# Autodesk Inventor assembly: 206.001.01_Schieberbetaetigung
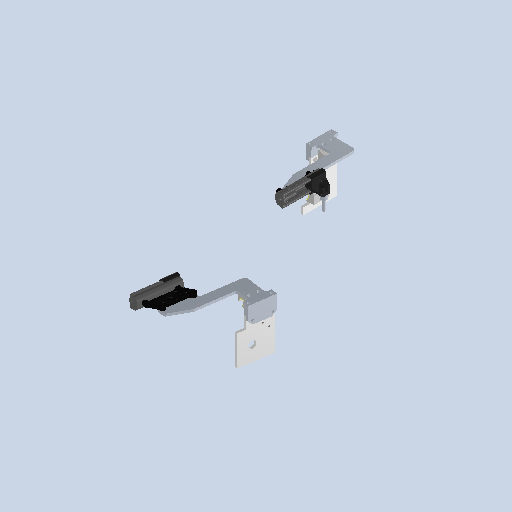
[picture p0: Inventor's stored thumbnail of the model, 512x512]
Saved by Autodesk Inventor 2022 (Build 260153000, 153)
## iProperties
Created: 2021-11-14
Part Number: 206.001.01_Schieberbetaetigung
Document SubType Name: Assembly
Designer: Oliver Ungerer
KODE_ZEICHNUNGSNUMMER: TFVEM_110M
BENENNUNG: Fuehrung Schieber
BEARBEITER_NAME: Ungerer O.
MASSE: 2.190774
PDMREV: 0.0+
PDMRL: Entwicklung
PROI_REVISION: 0
PROI_VERSION: 0+
PROI_RELEASE: Entwicklung
PTC_MODIFIED: True
PROI_CREATED_BY: Kantioler_adm
PROI_CREATED_ON: 07.03.2008 12:11:19
PROI_LOCATION: Root-Ordner/Pro_stds/Start_Files
MATERIALART: -
EINHEIT: ST
HERSTELLER_PREIS: 0.0
PRUEFER_NAME: Uo
PTC_ORGANIZATION_ID: Durst
PTC_WM_REVISION: 0
PTC_WM_ITERATION: 0
PTC_WM_VERSION: 0.0
PTC_WM_LIFECYCLE_STATE: Entwicklung
PTC_WM_LIFECYCLE: 02 Durst
PTC_WM_CREATED_BY: Oliver Ungerer (oungerer: Durst)
PTC_WM_CREATED_ON: 01.08.21
PTC_WM_MODIFIED_BY: Oliver Ungerer (oungerer: Durst)
PTC_WM_MODIFIED_ON: 01.08.21
AEND_INDEX: 0
VERSION: 0
STATUS: 0.0
Author: Oliver Ungerer
## Documents named in this file (11)
- C:\Users\kaebi\OneDrive - mci4me.at\03_MCI Master\4.Semester_SS2022\Masterarbeit\Software\CAD_TeachingFactory\206.002.01_Schieberbetaetigung.iam
- C:\Users\kaebi\OneDrive - mci4me.at\03_MCI Master\4.Semester_SS2022\Masterarbeit\Software\CAD_TeachingFactory\106.016.01_Schienenfuehrung.ipt
- C:\Users\kaebi\OneDrive - mci4me.at\03_MCI Master\4.Semester_SS2022\Masterarbeit\Software\CAD_TeachingFactory\106.019.01_Distanzplatte.ipt
- C:\Users\kaebi\OneDrive - mci4me.at\03_MCI Master\4.Semester_SS2022\Masterarbeit\Software\CAD_TeachingFactory\106.018.01_Schieberelement_oben.ipt
- C:\Users\kaebi\OneDrive - mci4me.at\03_MCI Master\4.Semester_SS2022\Masterarbeit\Software\CAD_TeachingFactory\106.020.01_Winkelaufnahme_Schwert_unten.ipt
- C:\Users\kaebi\OneDrive - mci4me.at\03_MCI Master\4.Semester_SS2022\Masterarbeit\Software\CAD_TeachingFactory\106.030.01_Schwert_oben.ipt
- C:\Users\kaebi\OneDrive - mci4me.at\03_MCI Master\4.Semester_SS2022\Masterarbeit\Software\CAD_TeachingFactory\106.033.01_Schwert_unten.ipt
- C:\Users\kaebi\OneDrive - mci4me.at\03_MCI Master\4.Semester_SS2022\Masterarbeit\Software\CAD_TeachingFactory\206.003.02_Kraftlimitierung.iam
- C:\Users\kaebi\OneDrive - mci4me.at\03_MCI Master\4.Semester_SS2022\Masterarbeit\Software\CAD_TeachingFactory\206.004.02_Kraftlimitierung.iam
- C:\Users\kaebi\OneDrive - mci4me.at\03_MCI Master\4.Semester_SS2022\Masterarbeit\Software\CAD_TeachingFactory\106.035.01_Distanzbolzen_gross.ipt
- C:\Users\kaebi\OneDrive - mci4me.at\03_MCI Master\4.Semester_SS2022\Masterarbeit\Software\CAD_TeachingFactory\106.034.01_Schieberelement_unten.ipt
## Components (15 placed, 10 different names)
1. 106.019.01_Distanzplatte — Passend:18, Passend:29, Passend:77, Passend:78, Passend:79
2. 106.019.01_Distanzplatte:1 — Passend:26, Passend:75, Passend:76, Passend:100, Passend:101
3. 106.035.01_Distanzbolzen_gross — Passend:59, Passend:60
4. 106.016.01_Schienenfuehrung:5 — Passend:97
5. 106.016.01_Schienenfuehrung:6 — Passend:98, Passend:99
6. 106.034.01_Schieberelement_unten:2 — Passend:97, Passend:98, Passend:99
7. 106.020.01_Winkelaufnahme_Schwert_unten:3
8. 106.033.01_Schwert_unten:2
9. 206.003.02_Kraftlimitierung:2 [sub-assembly]
10. 106.016.01_Schienenfuehrung — Passend:18, Passend:77, Passend:78
11. 106.016.01_Schienenfuehrung:1 — Passend:26, Passend:75, Passend:76, Passend:80
12. 106.018.01_Schieberelement_oben — Passend:29, Passend:36, Passend:37, Passend:38, Passend:50, Passend:79, Passend:80, Passend:83, Passend:84, Passend:100, Passend:101
13. 106.020.01_Winkelaufnahme_Schwert_unten — Passend:36, Passend:37, Passend:38, Passend:42, Passend:43, Passend:44
14. 106.030.01_Schwert_oben — Passend:42, Passend:43, Passend:44
15. 206.004.02_Kraftlimitierung [sub-assembly] — Passend:50, Passend:59, Passend:60, Passend:83, Passend:84
## Relationships (37: Mate 37)
- Passend:18 [Mate]: 106.019.01_Distanzplatte ↔ 106.016.01_Schienenfuehrung
- Passend:26 [Mate]: 106.019.01_Distanzplatte:1 ↔ 106.016.01_Schienenfuehrung:1
- Passend:29 [Mate]: 106.019.01_Distanzplatte ↔ 106.018.01_Schieberelement_oben
- Passend:36 [Mate]: 106.018.01_Schieberelement_oben ↔ 106.020.01_Winkelaufnahme_Schwert_unten
- Passend:37 [Mate]: 106.018.01_Schieberelement_oben ↔ 106.020.01_Winkelaufnahme_Schwert_unten
- Passend:38 [Mate]: 106.018.01_Schieberelement_oben ↔ 106.020.01_Winkelaufnahme_Schwert_unten
- Passend:42 [Mate]: 106.020.01_Winkelaufnahme_Schwert_unten ↔ 106.030.01_Schwert_oben
- Passend:43 [Mate]: 106.020.01_Winkelaufnahme_Schwert_unten ↔ 106.030.01_Schwert_oben
- Passend:44 [Mate]: 106.020.01_Winkelaufnahme_Schwert_unten ↔ 106.030.01_Schwert_oben
- Passend:50 [Mate]: 106.018.01_Schieberelement_oben ↔ 206.004.02_Kraftlimitierung
- Passend:59 [Mate]: 106.035.01_Distanzbolzen_gross ↔ 206.004.02_Kraftlimitierung
- Passend:60 [Mate]: 106.035.01_Distanzbolzen_gross ↔ 206.004.02_Kraftlimitierung
- Passend:75 [Mate]: 106.019.01_Distanzplatte:1 ↔ 106.016.01_Schienenfuehrung:1
- Passend:76 [Mate]: 106.019.01_Distanzplatte:1 ↔ 106.016.01_Schienenfuehrung:1
- Passend:77 [Mate]: 106.019.01_Distanzplatte ↔ 106.016.01_Schienenfuehrung
- Passend:78 [Mate]: 106.019.01_Distanzplatte ↔ 106.016.01_Schienenfuehrung
- Passend:79 [Mate]: 106.019.01_Distanzplatte ↔ 106.018.01_Schieberelement_oben
- Passend:80 [Mate]: 106.016.01_Schienenfuehrung:1 ↔ 106.018.01_Schieberelement_oben
- Passend:83 [Mate]: 106.018.01_Schieberelement_oben ↔ 206.004.02_Kraftlimitierung
- Passend:84 [Mate]: 106.018.01_Schieberelement_oben ↔ 206.004.02_Kraftlimitierung
- [Mate]: 106.016.01_Schienenfuehrung:6 ↔ 106.034.01_Schieberelement_unten:2
- [Mate]: 106.016.01_Schienenfuehrung:5 ↔ 106.034.01_Schieberelement_unten:2
- [Mate]: 106.034.01_Schieberelement_unten:2 ↔ 106.020.01_Winkelaufnahme_Schwert_unten:3
- [Mate]: 106.034.01_Schieberelement_unten:2 ↔ 106.020.01_Winkelaufnahme_Schwert_unten:3
- [Mate]: 106.034.01_Schieberelement_unten:2 ↔ 106.020.01_Winkelaufnahme_Schwert_unten:3
- [Mate]: 106.020.01_Winkelaufnahme_Schwert_unten:3 ↔ 106.033.01_Schwert_unten:2
- [Mate]: 106.020.01_Winkelaufnahme_Schwert_unten:3 ↔ 106.033.01_Schwert_unten:2
- [Mate]: 106.020.01_Winkelaufnahme_Schwert_unten:3 ↔ 106.033.01_Schwert_unten:2
- [Mate]: 106.034.01_Schieberelement_unten:2 ↔ 206.003.02_Kraftlimitierung:2
- [Mate]: 106.016.01_Schienenfuehrung:5 ↔ 106.034.01_Schieberelement_unten:2
- [Mate]: 106.034.01_Schieberelement_unten:2 ↔ 206.003.02_Kraftlimitierung:2
- [Mate]: 106.034.01_Schieberelement_unten:2 ↔ 206.003.02_Kraftlimitierung:2
- Passend:97 [Mate]: 106.016.01_Schienenfuehrung:5 ↔ 106.034.01_Schieberelement_unten:2
- Passend:98 [Mate]: 106.016.01_Schienenfuehrung:6 ↔ 106.034.01_Schieberelement_unten:2
- Passend:99 [Mate]: 106.016.01_Schienenfuehrung:6 ↔ 106.034.01_Schieberelement_unten:2
- Passend:100 [Mate]: 106.019.01_Distanzplatte:1 ↔ 106.018.01_Schieberelement_oben
- Passend:101 [Mate]: 106.019.01_Distanzplatte:1 ↔ 106.018.01_Schieberelement_oben
## Named parameters: d96_d84 = 0 mm, d97_d92 = 0 mm, d98_d93 = 0 mm, d99_d44 = 0 mm, d100_d45 = 0 mm, d101_d46 = 0 mm, d102_d52 = 0 mm, d103_d36 = 0 mm, d104_d37 = 0 mm, d105_d38 = 0 mm, d106_d39 = 0 mm, d107_d40 = 0 mm
